# Autodesk Inventor assembly: ControlBoard
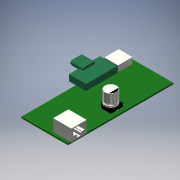
[picture p0: Inventor's stored thumbnail of the model, 180x180]
Saved by Autodesk Inventor 2016 (Build 200138000, 138)
## iProperties
Created: 2016-08-11
Part Number: ControlBoard
Document SubType Name: Assembly
Designer: jfixelle
Author: jfixelle
## Documents named in this file (5)
- E:\jfixelle\Documents\APC\GitRepo\Control\IAM\ControlBoard.iam
- E:\jfixelle\Documents\APC\GitRepo\Control\IAM\ControlBoard.ipt
- E:\jfixelle\Documents\APC\GitRepo\PCB_Libs\3DParts\RJE051AA1310.ipt
- E:\jfixelle\Documents\APC\GitRepo\PCB_Libs\3DParts\SMTElectro13x13x16.ipt
- E:\jfixelle\Documents\APC\GitRepo\PCB_Libs\3DParts\H11L1M.ipt
## Components (4 placed, 4 different names)
1. ControlBoard:1 — Mate:1, Mate:2, Flush:1, Flush:2, Mate:3
2. RJE051AA1310:1 — Mate:2, Flush:1, Flush:2
3. SMTElectro13x13x16:1 — Mate:3
4. H11L1M:1 — Mate:1
## Relationships (5: Mate 3, Flush 2)
- Mate:1: ControlBoard:1 ↔ H11L1M:1
- Mate:2: ControlBoard:1 ↔ RJE051AA1310:1
- Flush:1 (-0.635 mm): ControlBoard:1 ↔ RJE051AA1310:1
- Flush:2 (2.794 mm): ControlBoard:1 ↔ RJE051AA1310:1
- Mate:3: ControlBoard:1 ↔ SMTElectro13x13x16:1
